# Autodesk Inventor assembly: Neck
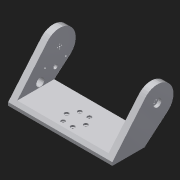
[picture p0: Inventor's stored thumbnail of the model, 180x180]
Saved by Autodesk Inventor 2017 SP1 (Build 210196100, 196)
## iProperties
Created: 2018-03-03
Part Number: Neck
Document SubType Name: Assembly
Designer: Zach
Author: Zach
## Documents named in this file (2)
- C:\Users\Zach\Documents\GitHub\tr1_description\meshes\Visual Assembly\Neck.iam
- C:\Users\Zach\Desktop\Neck.ipt
## Components (1 placed, 1 different names)
1. Neck:1 — Flush:1, Angle:1, Mate:1, Mate:2
## Relationships (4: Mate 2, Flush 1, Angle 1)
- Flush:1 (-10 mm): Neck:1
- Angle:1 (0 deg): Neck:1
- Mate:1 (142.5 mm): Neck:1
- Mate:2: Neck:1
